# Autodesk Inventor assembly: Butterfly Drive Module
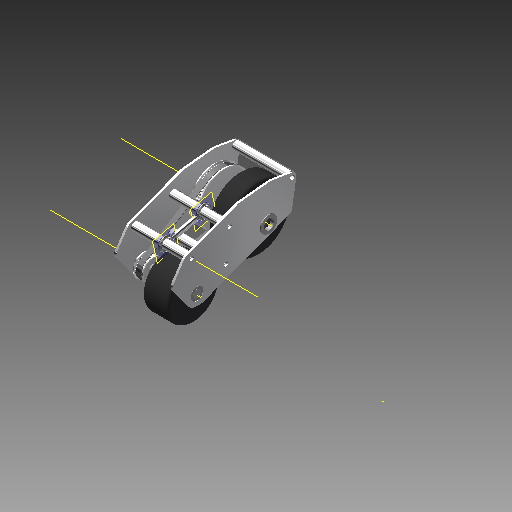
[picture p0: Inventor's stored thumbnail of the model, 512x512]
Saved by Autodesk Inventor 2019 (Build 230136000, 136)
## iProperties
Created: 2019-10-18
Part Number: Butterfly Drive Module
Document SubType Name: Assembly
Designer: admin
Author: admin
## Documents named in this file (11)
- C:\Users\Mark\Desktop\7738 Helion Engineering\7738-CAD-prep\Butterfly drive\Butterfly Drive Module.iam
- C:\Users\Mark\Desktop\7738 Helion Engineering\7738-CAD-prep\Butterfly drive\100mm Mecanum StandIn.ipt
- C:\Users\Mark\Desktop\7738 Helion Engineering\7738-CAD-prep\Butterfly drive\100mm Traction Wheel StandIn.ipt
- C:\Users\Mark\Desktop\7738 Helion Engineering\7738-CAD-prep\Butterfly drive\Butterfly Drive Module\Design Accelerator\Synchronous Belts Transmission3.iam
- C:\Users\Mark\Desktop\7738 Helion Engineering\7738-CAD-prep\Butterfly drive\Module Plate 1.ipt
- C:\Users\Mark\Desktop\7738 Helion Engineering\7738-CAD-prep\Butterfly drive\Connector.ipt
- C:\Users\Mark\Desktop\7738 Helion Engineering\7738-CAD-prep\Butterfly drive\F6004.ipt
- C:\Users\Mark\Desktop\7738 Helion Engineering\7738-CAD-prep\Butterfly drive\F6802.ipt
- C:\Users\Mark\Desktop\7738 Helion Engineering\7738-CAD-prep\Butterfly drive\Butterfly Drive Module\Design Accelerator\Shaft1.iam
- C:\Users\Mark\Desktop\7738 Helion Engineering\7738-CAD-prep\Butterfly drive\M6GBTeye.ipt
- C:\Users\Mark\Desktop\7738 Helion Engineering\7738-CAD-prep\Butterfly drive\Butterfly Drive Module\Design Accelerator\Shaft3.iam
## Components (17 placed, 9 different names)
1. Connector:1 — Mate:34, Mate:49, Mate:64, Mate:66
2. 100mm Mecanum StandIn:1 — Flush:1, Mate:5, Angle:1, Mate:37, Mate:42
3. 100mm Traction Wheel StandIn:1 — Mate:4, Flush:1, Mate:6
4. Synchronous Belts Transmission:1 [sub-assembly] — Mate:5, Mate:6, Mate:37, Mate:40, Mate:41, Angle:2
5. Module Plate 1:1 — Mate:33, Flush:2, Flush:3, Mate:39, Mate:41, Mate:42, Mate:43, Mate:44, Mate:45, Mate:46, Mate:52, Mate:55, Mate:57, Mate:58, Mate:64, Mate:65, Mate:66, Mate:67
6. Module Plate 1:2 — Mate:33, Flush:2, Flush:3, Mate:50, Mate:53, Mate:54, Mate:59, Mate:60, Angle:2
7. F6804:1 — Mate:59, Mate:60
8. F6804:2 — Mate:57, Mate:58
9. F6802:1 — Mate:53, Mate:54
10. F6802:2 — Mate:52, Mate:55, Mate:61, Flush:4
11. Connector:2 — Mate:43, Mate:44
12. Shaft:1 [sub-assembly] — Mate:61, Flush:4
13. Connector:3 — Mate:45, Mate:46
14. M6GBTeye:1 — Mate:47, Mate:49, Mate:50, Mate:51, Mate:62
15. M6GBTeye:2 — Mate:47, Mate:48, Mate:63
16. Connector:4 — Mate:48, Mate:65, Mate:67
17. Shaft:2 [sub-assembly] — Mate:62, Mate:63
## Relationships (40: Mate 34, Flush 4, Angle 2)
- Mate:4: 100mm Traction Wheel StandIn:1
- Flush:1 (10.5 mm): 100mm Mecanum StandIn:1 ↔ 100mm Traction Wheel StandIn:1
- Mate:5: 100mm Mecanum StandIn:1 ↔ Synchronous Belts Transmission:1
- Mate:6: 100mm Traction Wheel StandIn:1 ↔ Synchronous Belts Transmission:1
- Angle:1 (90 deg): 100mm Mecanum StandIn:1
- Mate:33 (105 mm): Module Plate 1:1 ↔ Module Plate 1:2
- Mate:34: Connector:1
- Flush:2: Module Plate 1:1 ↔ Module Plate 1:2
- Flush:3: Module Plate 1:1 ↔ Module Plate 1:2
- Mate:37 (2 mm): 100mm Mecanum StandIn:1 ↔ Synchronous Belts Transmission:1
- Mate:39: Module Plate 1:1
- Mate:40: Synchronous Belts Transmission:1
- Mate:41: Synchronous Belts Transmission:1 ↔ Module Plate 1:1
- Mate:42 (3.5 mm): 100mm Mecanum StandIn:1 ↔ Module Plate 1:1
- Mate:43: Module Plate 1:1 ↔ Connector:2
- Mate:44: Module Plate 1:1 ↔ Connector:2
- Mate:45: Module Plate 1:1 ↔ Connector:3
- Mate:46: Module Plate 1:1 ↔ Connector:3
- Mate:47: M6GBTeye:1 ↔ M6GBTeye:2
- Mate:48: M6GBTeye:2 ↔ Connector:4
- Mate:49: Connector:1 ↔ M6GBTeye:1
- Mate:50 (58.5 mm): Module Plate 1:2 ↔ M6GBTeye:1
- Mate:51: M6GBTeye:1
- Mate:52: Module Plate 1:1 ↔ F6802:2
- Mate:53: Module Plate 1:2 ↔ F6802:1
- Mate:54 (0.2 mm): Module Plate 1:2 ↔ F6802:1
- Mate:55 (0.2 mm): Module Plate 1:1 ↔ F6802:2
- Mate:57: Module Plate 1:1 ↔ F6804:2
- Mate:58 (0.2 mm): Module Plate 1:1 ↔ F6804:2
- Mate:59: Module Plate 1:2 ↔ F6804:1
- Mate:60 (0.2 mm): Module Plate 1:2 ↔ F6804:1
- Mate:61: F6802:2 ↔ Shaft:1
- Flush:4 (-0.2 mm): F6802:2 ↔ Shaft:1
- Mate:62: M6GBTeye:1 ↔ Shaft:2
- Mate:63 (3 mm): M6GBTeye:2 ↔ Shaft:2
- Mate:64: Connector:1 ↔ Module Plate 1:1
- Mate:65: Module Plate 1:1 ↔ Connector:4
- Mate:66 (0.3 mm): Connector:1 ↔ Module Plate 1:1
- Mate:67 (0.3 mm): Module Plate 1:1 ↔ Connector:4
- Angle:2 (0 deg): Synchronous Belts Transmission:1 ↔ Module Plate 1:2
